# Autodesk Inventor assembly: Pelvis
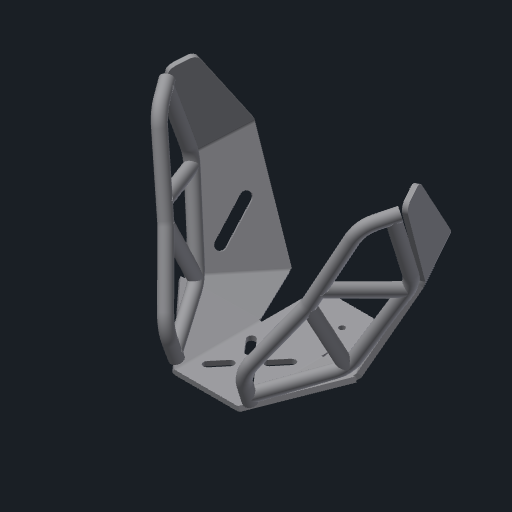
[picture p0: Inventor's stored thumbnail of the model, 512x512]
Saved by Autodesk Inventor 2025.2 (Build 292293000, 293)
## iProperties
Created: 2020-05-05
Part Number: Pelvis
Document SubType Name: Assembly
Designer: valer
Author: valer
## Documents named in this file (3)
- C:\Users\valer\Desktop\str1ker\cad\Pelvis.iam
- C:\Users\valer\Desktop\str1ker\cad\PelvisWing.ipt
- C:\Users\valer\Desktop\str1ker\cad\SpineRoot.ipt
## Components (3 placed, 2 different names)
1. PelvisWing:3 — Flush:3
2. PelvisWing:4 — Mate:1
3. SpineRoot:1 — Flush:1, Flush:2, Mate:1, Flush:3, Mate:2
## Relationships (5: Flush 3, Mate 2)
- Flush:1: SpineRoot:1
- Flush:2: SpineRoot:1
- Mate:1: PelvisWing:4 ↔ SpineRoot:1
- Flush:3: PelvisWing:3 ↔ SpineRoot:1
- Mate:2: SpineRoot:1
